# Autodesk Inventor assembly: ForeArm
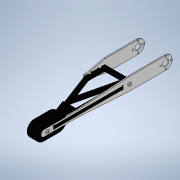
[picture p0: Inventor's stored thumbnail of the model, 180x180]
Saved by Autodesk Inventor 2020 (Build 240168000, 168)
## iProperties
Created: 2016-05-04
Part Number: ForeArm
Document SubType Name: Assembly
Designer: hiroaki
Mass: 59.7567 g
Surface Area: 275.043 cm^2
Volume: 46.6042 cm^3
Density: 1.28222 g/cm^3
Author: hiroaki
## Documents named in this file (8)
- C:\Users\Masato\Documents\Inventor\CIT Brains_Inventor\OpenPlatform_ver3_0\UpperBody\Arm\ForeArm.iam
- C:\Users\Masato\Documents\Inventor\CIT Brains_Inventor\OpenPlatform_ver3_0\UpperBody\Arm\ForeArm_outside_frame.ipt
- C:\Users\Masato\Documents\Inventor\CIT Brains_Inventor\OpenPlatform_ver3_0\UpperBody\Arm\ForeArm_diagonal.ipt
- C:\Users\Masato\Documents\Inventor\CIT Brains_Inventor\OpenPlatform_ver3_0\UpperBody\Arm\ForeArm_inside_frame.ipt
- C:\Users\Masato\Documents\Inventor\CIT Brains_Inventor\OpenPlatform_ver3_0\Ready_Made\Screw\M3-6.ipt
- C:\Users\Masato\Documents\Inventor\CIT Brains_Inventor\OpenPlatform_ver3_0\Ready_Made\Screw\M3-10.ipt
- C:\Users\Masato\Documents\Inventor\CIT Brains_Inventor\OpenPlatform_ver3_0\Ready_Made\UD-43040.ipt
- C:\Users\Masato\Documents\Inventor\CIT Brains_Inventor\OpenPlatform_ver3_0\UpperBody\Arm\Hand.ipt
## Components (9 placed, 7 different names)
1. ForeArm_diagonal:1 — メイト:1, メイト:2, フラッシュ:1, 挿入:3, 挿入:4, 挿入:5, 挿入:6, 角度:1, 挿入:12
2. ForeArm_outside_frame:1 — 挿入:3, 挿入:4, 挿入:7, 挿入:10
3. ForeArm_inside_frame:1 — 挿入:5, 挿入:6, 挿入:8, 挿入:9
4. M3-6:1 — 挿入:7
5. M3-6:2 — 挿入:8
6. M3-6:3 — 挿入:9
7. M3-10:1 — 挿入:10
8. UD-43040:1 — 挿入:11
9. Hand:1 — 角度:1, 挿入:12, 挿入:11
## Relationships (14: Insert 10, Mate 2, Flush 1, Angle 1)
- メイト:1 [Mate]: ForeArm_diagonal:1
- メイト:2 [Mate]: ForeArm_diagonal:1
- フラッシュ:1 [Flush]: ForeArm_diagonal:1
- 挿入:3 [Insert]: ForeArm_diagonal:1 ↔ ForeArm_outside_frame:1
- 挿入:4 [Insert]: ForeArm_diagonal:1 ↔ ForeArm_outside_frame:1
- 挿入:5 [Insert]: ForeArm_diagonal:1 ↔ ForeArm_inside_frame:1
- 挿入:6 [Insert]: ForeArm_diagonal:1 ↔ ForeArm_inside_frame:1
- 挿入:7 [Insert]: ForeArm_outside_frame:1 ↔ M3-6:1
- 挿入:8 [Insert]: ForeArm_inside_frame:1 ↔ M3-6:2
- 挿入:9 [Insert]: ForeArm_inside_frame:1 ↔ M3-6:3
- 挿入:10 [Insert]: ForeArm_outside_frame:1 ↔ M3-10:1
- 挿入:11 [Insert]: UD-43040:1 ↔ Hand:1
- 角度:1 [Angle] (0 deg): ForeArm_diagonal:1 ↔ Hand:1
- 挿入:12 [Insert] (0.25 mm): ForeArm_diagonal:1 ↔ Hand:1
